# Autodesk Inventor assembly: VertDamage
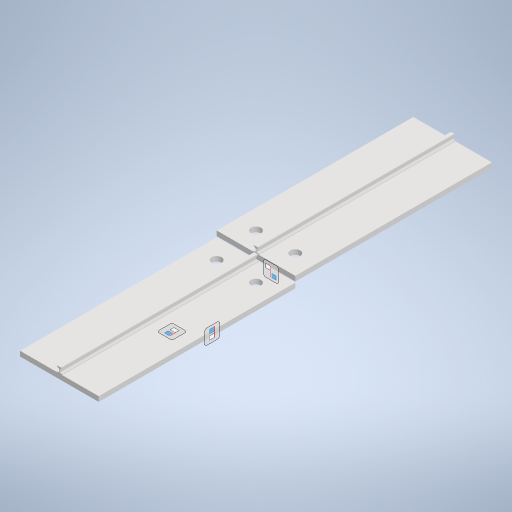
[picture p0: Inventor's stored thumbnail of the model, 512x512]
Saved by Autodesk Inventor 2023 (Build 270158030, 158C)
## iProperties
Created: 2023-02-14
Part Number: VertDamage
Document SubType Name: Assembly
Designer: jeremyy
Author: jeremyy
## Documents named in this file (2)
- \\andrew.ad.cmu.edu\users\users1\jeremyy\Documents\Inventor\CMU Bridge\New folder\Figs\VertDamage.iam
- \\andrew.ad.cmu.edu\users\users1\jeremyy\Documents\Inventor\CMU Bridge\New folder\Figs\SideUndamaged.iam
## Components (2 placed, 1 different names)
1. SideUndamaged:1 [sub-assembly] — Mate:1, Flush:1, Flush:2
2. SideUndamaged:2 [sub-assembly] — Mate:1, Flush:1, Flush:2
## Relationships (3: Flush 2, Mate 1)
- Mate:1: SideUndamaged:1 ↔ SideUndamaged:2
- Flush:1 (-3.81 mm): SideUndamaged:1 ↔ SideUndamaged:2
- Flush:2: SideUndamaged:1 ↔ SideUndamaged:2
